# Autodesk Inventor assembly: Сборка1
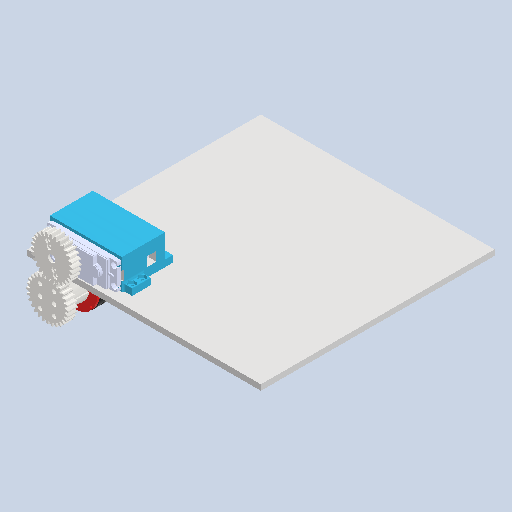
[picture p0: Inventor's stored thumbnail of the model, 512x512]
Saved by Autodesk Inventor 2022 (Build 260153000, 153)
## iProperties
Created: 2022-12-27
Part Number: Сборка1
Document SubType Name: Assembly
Designer: Pavel
Author: Pavel
## Documents named in this file (9)
- F:\Новая папка\Сборка1.iam
- F:\Новая папка\мотор_плеча_1v2.ipt
- F:\Новая папка\Servo body.ipt
- F:\Новая папка\доска.ipt
- F:\Новая папка\двухопорный корпус.ipt
- F:\Новая папка\держалка подша.ipt
- F:\Новая папка\шестерня_2.ipt
- F:\Новая папка\шестерня_1.ipt
- F:\Новая папка\трубка.ipt
## Components (8 placed, 7 different names)
1. мотор_плеча_1v2:1 — Совмещение:1, Совмещение:2, Совмещение:3, Совмещение:4, Заподлицо:2
2. Servo body:1 — Совмещение:1, Совмещение:2, Совмещение:3, Заподлицо:1, Совмещение:14
3. доска:1 — Совмещение:4, Заподлицо:1, Заподлицо:2, Совмещение:5, Заподлицо:4, Совмещение:6
4. двухопорный корпус:1 — Совмещение:5, Заподлицо:4, Совмещение:10, Совмещение:15, Совмещение:16, Совмещение:17
5. держалка подша:1 — Совмещение:6, Совмещение:13, Совмещение:15, Совмещение:16, Совмещение:17
6. Цилиндрическое зубчатое зацепление2:1 — Совмещение:11, Совмещение:12, Совмещение:13
7. Цилиндрическое зубчатое зацепление2:2 — Совмещение:14
8. трубка:1 — Совмещение:10, Совмещение:11, Совмещение:12
## Relationships (17: Mate 14, Flush 3)
- Совмещение:1 [Mate]: мотор_плеча_1v2:1 ↔ Servo body:1
- Совмещение:2 [Mate]: мотор_плеча_1v2:1 ↔ Servo body:1
- Совмещение:3 [Mate]: мотор_плеча_1v2:1 ↔ Servo body:1
- Совмещение:4 [Mate]: мотор_плеча_1v2:1 ↔ доска:1
- Заподлицо:1 [Flush]: Servo body:1 ↔ доска:1
- Заподлицо:2 [Flush]: мотор_плеча_1v2:1 ↔ доска:1
- Совмещение:5 [Mate]: доска:1 ↔ двухопорный корпус:1
- Заподлицо:4 [Flush]: доска:1 ↔ двухопорный корпус:1
- Совмещение:6 [Mate]: доска:1 ↔ держалка подша:1
- Совмещение:10 [Mate]: двухопорный корпус:1 ↔ трубка:1
- Совмещение:11 [Mate]: Цилиндрическое зубчатое зацепление2:1 ↔ трубка:1
- Совмещение:12 [Mate] (0.2 mm): Цилиндрическое зубчатое зацепление2:1 ↔ трубка:1
- Совмещение:13 [Mate] (0.1 mm): держалка подша:1 ↔ Цилиндрическое зубчатое зацепление2:1
- Совмещение:14 [Mate]: Servo body:1 ↔ Цилиндрическое зубчатое зацепление2:2
- Совмещение:15 [Mate]: двухопорный корпус:1 ↔ держалка подша:1
- Совмещение:16 [Mate]: двухопорный корпус:1 ↔ держалка подша:1
- Совмещение:17 [Mate]: двухопорный корпус:1 ↔ держалка подша:1
